# Autodesk Inventor assembly: Washing Machine Assembly
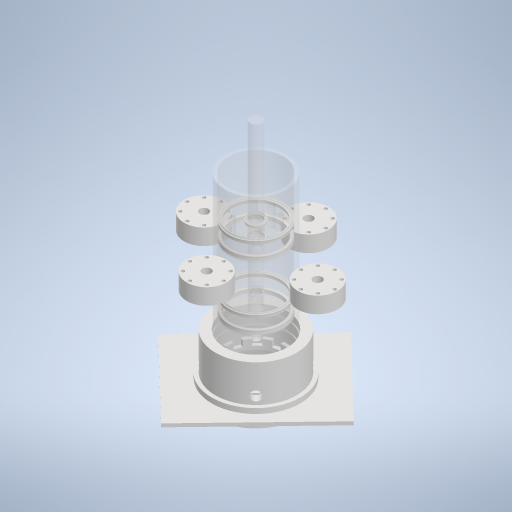
[picture p0: Inventor's stored thumbnail of the model, 512x512]
Saved by Autodesk Inventor 2024 (Build 280153000, 153)
## iProperties
Created: 2024-04-17
Part Number: Washing Machine Assembly
Document SubType Name: Assembly
Designer: Tommy Rohmann
Author: Tommy Rohmann
## Documents named in this file (7)
- C:\Users\Tommy Rohmann\Documents\Repositories\Microgravity-Press-Washing-Machine\Sub-System Design and Documentation\Washing Machine Assembly.iam
- C:\Users\Tommy Rohmann\Documents\Repositories\Microgravity-Press-Washing-Machine\Sub-System Design and Documentation\3 Wash Chamber Assembly\Wash Chamber Assembly.iam
- C:\Users\Tommy Rohmann\Documents\Repositories\Microgravity-Press-Washing-Machine\Sub-System Design and Documentation\2 Chamber Top Piston Assembly\Chamber Top Assembly.iam
- C:\Users\Tommy Rohmann\Documents\Repositories\Microgravity-Press-Washing-Machine\Sub-System Design and Documentation\1 Piston Assembly\Piston Assembly.iam
- C:\Users\Tommy Rohmann\Documents\Repositories\Microgravity-Press-Washing-Machine\Sub-System Design and Documentation\4 Structure and Drive Train Assembly\1 Bottom Frame Base 1.ipt
- C:\Users\Tommy Rohmann\Documents\Repositories\Microgravity-Press-Washing-Machine\Sub-System Design and Documentation\4 Structure and Drive Train Assembly\2 Bottom Frame Base 2.ipt
- C:\Users\Tommy Rohmann\Documents\Repositories\Microgravity-Press-Washing-Machine\Sub-System Design and Documentation\4 Structure and Drive Train Assembly\7 Load Cell.ipt
## Components (11 placed, 6 different names)
1. Wash Chamber Assembly:1 [sub-assembly] — Mate:1, Mate:2, Mate:4, Mate:7, Mate:9, Mate:10, Mate:11, Mate:13
2. Chamber Top Assembly:1 [sub-assembly] — Mate:3
3. Piston Assembly:1 [sub-assembly] — Mate:1, Mate:2, Mate:3
4. 1 Bottom Frame Base 1:1 — Mate:8, Mate:9, Mate:10, Mate:14
5. 2 Bottom Frame Base 2:1 — Mate:11, Mate:12, Mate:15, Flush:1
6. 1 Bottom Frame Base 1:2 — Mate:4, Mate:7, Mate:8, Mate:12, Flush:1
7. 2 Bottom Frame Base 2:2 — Mate:13, Mate:14, Mate:15
8. 7 Load Cell:1
9. 7 Load Cell:2
10. 7 Load Cell:3
11. 7 Load Cell:4
## Relationships (14: Mate 13, Flush 1)
- Mate:1: Wash Chamber Assembly:1 ↔ Piston Assembly:1
- Mate:2: Wash Chamber Assembly:1 ↔ Piston Assembly:1
- Mate:3: Chamber Top Assembly:1 ↔ Piston Assembly:1
- Mate:4: Wash Chamber Assembly:1 ↔ 1 Bottom Frame Base 1:2
- Mate:7: Wash Chamber Assembly:1 ↔ 1 Bottom Frame Base 1:2
- Mate:8: 1 Bottom Frame Base 1:1 ↔ 1 Bottom Frame Base 1:2
- Mate:9: Wash Chamber Assembly:1 ↔ 1 Bottom Frame Base 1:1
- Mate:10: Wash Chamber Assembly:1 ↔ 1 Bottom Frame Base 1:1
- Mate:11: Wash Chamber Assembly:1 ↔ 2 Bottom Frame Base 2:1
- Mate:12: 2 Bottom Frame Base 2:1 ↔ 1 Bottom Frame Base 1:2
- Mate:13: Wash Chamber Assembly:1 ↔ 2 Bottom Frame Base 2:2
- Mate:14: 1 Bottom Frame Base 1:1 ↔ 2 Bottom Frame Base 2:2
- Mate:15: 2 Bottom Frame Base 2:1 ↔ 2 Bottom Frame Base 2:2
- Flush:1: 2 Bottom Frame Base 2:1 ↔ 1 Bottom Frame Base 1:2
